# Autodesk Inventor assembly: v1_assem
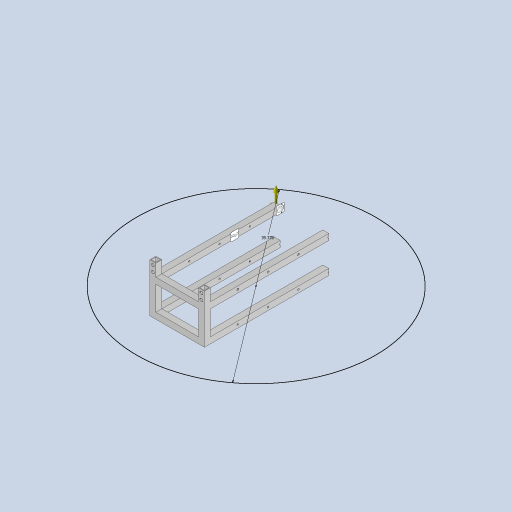
[picture p0: Inventor's stored thumbnail of the model, 512x512]
Saved by Autodesk Inventor 2023 (Build 270158030, 158C)
## iProperties
Created: 2022-07-26
Part Number: v1_assem
Document SubType Name: Assembly
Designer: kumpu
Mass: 36098.2 g
Surface Area: 53416.4 cm^2
Volume: 78394.7 cm^3
Density: 0.460468 g/cm^3
Author: kumpu
## Documents named in this file (13)
- C:\Users\kumpu\Documents\SBU\CAD\SBRT\Robocup Rescue\Drive\v1\v1_loading.iam
- C:\Users\kumpu\Documents\SBU\CAD\SBRT\Robocup Rescue\Drive\v1\Placeholder_ChassisMain.ipt
- C:\Users\kumpu\Documents\SBU\CAD\SBRT\Robocup Rescue\Drive\v1\T-Slotted Framing.ipt
- C:\Users\kumpu\Documents\Other Projects\vtol\95412A316_18-8 Stainless Steel Threaded Rod.ipt
- C:\Users\kumpu\Documents\Other Projects\vtol\91259A585_Alloy Steel Shoulder Screw.ipt
- C:\Users\kumpu\Documents\SBU\CAD\SBRT\Robocup Rescue\Drive\v1\96505A116_Steel Oversized Washer.ipt
- C:\Users\kumpu\Documents\SBU\CAD\SBRT\Robocup Rescue\Drive\v1\compressionSpacer.ipt
- C:\Users\kumpu\Documents\SBU\CAD\SBRT\Robocup Rescue\Drive\v1\v1_loading\AIP\FEA\e7yoolrts.fins
- C:\Users\kumpu\Documents\SBU\CAD\SBRT\Robocup Rescue\Drive\v1\v1_loading\AIP\FEA\e7yoolrts.fsat
- C:\Users\kumpu\Documents\SBU\CAD\SBRT\Robocup Rescue\Drive\v1\v1_loading\AIP\FEA\e7yoolrts.ftes
- C:\Users\kumpu\Documents\SBU\CAD\SBRT\Robocup Rescue\Drive\v1\v1_loading\AIP\FEA\e7yoolrts.fwiz
- C:\Users\kumpu\Documents\SBU\CAD\SBRT\Robocup Rescue\Drive\v1\v1_loading\AIP\FEA\e7yoolrvk.fmsh
- C:\Users\kumpu\Documents\SBU\CAD\SBRT\Robocup Rescue\Drive\v1\v1_loading\AIP\FEA\e7yoolrvl.fres
## Components (9 placed, 6 different names)
1. 95412A316_18-8 Stainless Steel Threaded Rod:1 — Mate:96, Flush:103
2. 91259A585_Alloy Steel Shoulder Screw:1 — Mate:94, Mate:95, Insert:23, Mate:97
3. 96505A116_Steel Oversized Washer:1 — Insert:23
4. compressionSpacer:1 — Mate:97, Angle:1, Mate:98
5. Placeholder_ChassisMain:1 — Mate:17, Mate:18, Flush:5, Mate:85, Mate:86, Flush:98, Mate:94, Mate:95, Mate:96, Flush:103, Angle:1, Mate:98
6. T-Slotted Framing:1 — Mate:85, Mate:86, Flush:98
7. T-Slotted Framing:2
8. T-Slotted Framing:3
9. T-Slotted Framing:4
## Component patterns: (4 elements, first: T-Slotted Framing:1)
## Relationships (15: Mate 9, Flush 4, Insert 1, Angle 1)
- Flush:2 (-31.75 mm)
- Mate:17: Placeholder_ChassisMain:1
- Mate:18: Placeholder_ChassisMain:1
- Flush:5: Placeholder_ChassisMain:1
- Mate:85 (101.6 mm): Placeholder_ChassisMain:1 ↔ T-Slotted Framing:1
- Mate:86: Placeholder_ChassisMain:1 ↔ T-Slotted Framing:1
- Flush:98: Placeholder_ChassisMain:1 ↔ T-Slotted Framing:1
- Mate:94: 91259A585_Alloy Steel Shoulder Screw:1 ↔ Placeholder_ChassisMain:1
- Mate:95: 91259A585_Alloy Steel Shoulder Screw:1 ↔ Placeholder_ChassisMain:1
- Mate:96: 95412A316_18-8 Stainless Steel Threaded Rod:1 ↔ Placeholder_ChassisMain:1
- Flush:103 (-12.7 mm): 95412A316_18-8 Stainless Steel Threaded Rod:1 ↔ Placeholder_ChassisMain:1
- Insert:23: 91259A585_Alloy Steel Shoulder Screw:1 ↔ 96505A116_Steel Oversized Washer:1
- Mate:97: 91259A585_Alloy Steel Shoulder Screw:1 ↔ compressionSpacer:1
- Angle:1 (0 deg): compressionSpacer:1 ↔ Placeholder_ChassisMain:1
- Mate:98: compressionSpacer:1 ↔ Placeholder_ChassisMain:1
## Named parameters: sa_0 = 9786.09
note: some values were not read from the file. Shown as the stored number, unit unknown: "sa_0".
